# Autodesk Inventor assembly: Assembly10
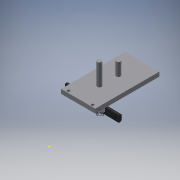
[picture p0: Inventor's stored thumbnail of the model, 180x180]
Saved by Autodesk Inventor 2019.4 (Build 234330000, 330)
## iProperties
Created: 2020-03-04
Part Number: Assembly10
Document SubType Name: Assembly
Designer: Niran
Author: Niran
## Documents named in this file (6)
- C:\Users\Niran\Desktop\sketch_jan26a\Canon parts\Assembly10.iam
- C:\Users\Niran\Desktop\sketch_jan26a\Canon parts\Part100.ipt
- C:\Users\Niran\Desktop\sketch_jan26a\Canon parts\VIRTUAL IMPLEMENTATION\rod2.ipt
- C:\Users\Niran\Desktop\sketch_jan26a\Canon parts\VIRTUAL IMPLEMENTATION\rod4.ipt
- C:\Users\Niran\Desktop\sketch_jan26a\Canon parts\VIRTUAL IMPLEMENTATION\gear_z18_m1.ipt
- C:\Users\Niran\Desktop\sketch_jan26a\Canon parts\VIRTUAL IMPLEMENTATION\Rack.ipt
## Components (6 placed, 5 different names)
1. Part100:1 — Rotational:1, Rigid:1
2. rod2:1 — Rotational:1, Rotational:2
3. rod2:2 — Rigid:1
4. rod4:1 — Rotational:2, Rotational:3
5. gear_z18_m1:1 — Rotational:3, Rotational:4
6. Rack:1 — Rotational:4
## Relationships (5: RevoluteJoint 4, WeldJoint 1)
- Rotational:1 [RevoluteJoint] (-50 mm): Part100:1 ↔ rod2:1
- Rigid:1 [WeldJoint] (30 mm): Part100:1 ↔ rod2:2
- Rotational:2 [RevoluteJoint]: rod2:1 ↔ rod4:1
- Rotational:3 [RevoluteJoint]: rod4:1 ↔ gear_z18_m1:1
- Rotational:4 [RevoluteJoint]: gear_z18_m1:1 ↔ Rack:1
